# Autodesk Inventor assembly: SensorA
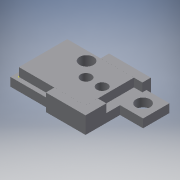
[picture p0: Inventor's stored thumbnail of the model, 180x180]
Saved by Autodesk Inventor 2018 (Build 220112000, 112)
## iProperties
Created: 2018-05-09
Part Number: SensorA
Document SubType Name: Assembly
Designer: s4321966
Author: s4321966
## Documents named in this file (3)
- H:\Inventor-Workspace\METR4901\Sensor Mount\SensorA.iam
- H:\Inventor-Workspace\METR4901\Sensor Mount\SensorMount.ipt
- H:\Inventor-Workspace\METR4901\Sensor Mount\SensorPCB.ipt
## Components (2 placed, 2 different names)
1. SensorMount:1 — Mate:1, Tangent:1
2. SensorPCB:1 — Mate:1, Tangent:1
## Relationships (2: Mate 1, Tangent 1)
- Mate:1: SensorMount:1 ↔ SensorPCB:1
- Tangent:1: SensorMount:1 ↔ SensorPCB:1
